# Autodesk Inventor assembly: Сборка1
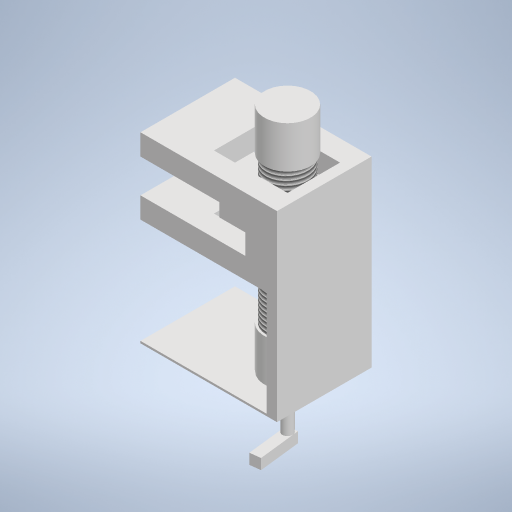
[picture p0: Inventor's stored thumbnail of the model, 512x512]
Saved by Autodesk Inventor 2023 (Build 270158000, 158)
## iProperties
Created: 2022-04-28
Part Number: Сборка1
Document SubType Name: Assembly
Designer: User
Author: User
## Documents named in this file (4)
- D:\Стойка\Механизм\Сборка1.iam
- D:\Стойка\Механизм\Вал штурвала.ipt
- D:\Стойка\Механизм\Деталь перемещение по резьбе.ipt
- D:\Стойка\Механизм\Стенка.ipt
## Components (3 placed, 3 different names)
1. Вал штурвала:1 — С поворотом:2, Цилиндрический:1
2. Деталь перемещение по резьбе:1 — Цилиндрический:1, Совмещение:1
3. Стенка:1 — С поворотом:2, Совмещение:1
## Relationships (3: RevoluteJoint 1, CylindricalJoint 1, Mate 1)
- С поворотом:2 [RevoluteJoint]: Вал штурвала:1 ↔ Стенка:1
- Цилиндрический:1 [CylindricalJoint]: Вал штурвала:1 ↔ Деталь перемещение по резьбе:1
- Совмещение:1 [Mate]: Деталь перемещение по резьбе:1 ↔ Стенка:1
